# Autodesk Inventor assembly: TheLightWithinYou-Assembly-V2
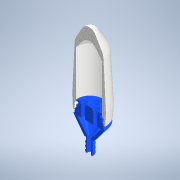
[picture p0: Inventor's stored thumbnail of the model, 180x180]
Saved by Autodesk Inventor 2021 (Build 250183000, 183)
## iProperties
Created: 2021-08-12
Part Number: TheLightWithinYou-Assembly-V2
Document SubType Name: Assembly
Designer: incep
Author: incep
## Documents named in this file (3)
- C:\Users\incep\Desktop\3D Printer Stuff\TheLightWithinYou\TheLightWithinYou-Assembly-V2.iam
- C:\Users\incep\Desktop\3D Printer Stuff\TheLightWithinYou\Bottom-Threaded-V2.ipt
- C:\Users\incep\Desktop\3D Printer Stuff\TheLightWithinYou\Upper-Threaded-v2.ipt
## Components (2 placed, 2 different names)
1. Bottom-Threaded-V2:1 — Mate:1, Mate:2
2. Upper-Threaded-v2:1 — Mate:1, Mate:2
## Relationships (2: Mate 2)
- Mate:1: Bottom-Threaded-V2:1 ↔ Upper-Threaded-v2:1
- Mate:2 (4 mm): Bottom-Threaded-V2:1 ↔ Upper-Threaded-v2:1
